# Autodesk Inventor assembly: TransmissionPuileyCenter
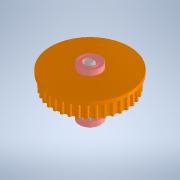
[picture p0: Inventor's stored thumbnail of the model, 180x180]
Saved by Autodesk Inventor 2022.2 (Build 262287000, 287)
## iProperties
Created: 2022-01-08
Part Number: TransmissionPuileyCenter
Document SubType Name: Assembly
Designer: Jochen
Author: Jochen
## Documents named in this file (5)
- D:\Projects\Lisbeth\CAD\Common\Motor\TransmissionPuileyCenter.iam
- D:\Projects\Lisbeth\CAD\Common\Motor\TransmissionPulleyCentreAxis.ipt
- D:\Projects\Lisbeth\CAD\Common\Motor\TransmissionCenterBigPulley.ipt
- D:\Projects\Lisbeth\CAD\Common\Motor\bearing_8_4_2_sbn_MR84VA.ipt
- D:\Projects\Lisbeth\CAD\Common\Washer\Washer m2.5.ipt
## Components (6 placed, 4 different names)
1. MotorBeltTensionerAxis:1 — Mate:2, Mate:3, Mate:10, Mate:13, Mate:18, Mate:21
2. Center Pulley T2.5:1 — Mate:21, Mate:22, Mate:23
3. bearing_8_4_2_sbn_MR84VA:1 — Mate:2, Mate:19
4. bearing_8_4_2_sbn_MR84VA:2 — Mate:3, Mate:12, Mate:18
5. Washer m2.5:1 — Mate:10, Mate:12, Mate:22
6. Washer m2.5:2 — Mate:13, Mate:19, Mate:23
## Relationships (10: Mate 10)
- Mate:2: MotorBeltTensionerAxis:1 ↔ bearing_8_4_2_sbn_MR84VA:1
- Mate:3: MotorBeltTensionerAxis:1 ↔ bearing_8_4_2_sbn_MR84VA:2
- Mate:10: MotorBeltTensionerAxis:1 ↔ Washer m2.5:1
- Mate:12: bearing_8_4_2_sbn_MR84VA:2 ↔ Washer m2.5:1
- Mate:13: MotorBeltTensionerAxis:1 ↔ Washer m2.5:2
- Mate:18: MotorBeltTensionerAxis:1 ↔ bearing_8_4_2_sbn_MR84VA:2
- Mate:19: bearing_8_4_2_sbn_MR84VA:1 ↔ Washer m2.5:2
- Mate:21: MotorBeltTensionerAxis:1 ↔ Center Pulley T2.5:1
- Mate:22: Center Pulley T2.5:1 ↔ Washer m2.5:1
- Mate:23: Center Pulley T2.5:1 ↔ Washer m2.5:2
